# Autodesk Inventor assembly: entero
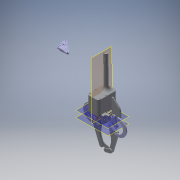
[picture p0: Inventor's stored thumbnail of the model, 180x180]
Saved by Autodesk Inventor 2018 (Build 220112000, 112)
## iProperties
Created: 2018-05-25
Part Number: entero
Document SubType Name: Assembly
Designer: vigus
Author: vigus
## Documents named in this file (8)
- C:\Users\vigus\Documents\gihug\hecatonquiros\cad_models\accesories\gripper\entero.iam
- C:\Users\vigus\Documents\gihug\hecatonquiros\cad_models\tools\gripper\serial_model_0dof\core_attachment.ipt
- C:\Users\vigus\Documents\gihug\hecatonquiros\cad_models\accesories\gripper\Imported Components\garra_pilar\garra_pilar.ipt
- C:\Users\vigus\Documents\gihug\hecatonquiros\cad_models\tools\gripper\serial_model_0dof\ScrewActuatorGripperCenter.ipt
- C:\Users\vigus\Documents\gihug\hecatonquiros\cad_models\tools\gripper\serial_model_0dof\gripper.ipt
- C:\Users\vigus\Documents\gihug\hecatonquiros\cad_models\accesories\gripper\garra_pilar_3.ipt
- C:\Users\vigus\Documents\gihug\hecatonquiros\cad_models\accesories\gripper\barra_tri.ipt
- C:\Users\vigus\Documents\gihug\hecatonquiros\cad_models\accesories\gripper\barra_triangulo.ipt
## Components (13 placed, 7 different names)
1. core_attachment:1 — Mate:2, Mate:3, Mate:13, Mate:14, Angle:1, Mate:32, Mate:42, Mate:43, Mate:52, Mate:53, Mate:55, Mate:56, Mate:69, Mate:70, Flush:1, Flush:2
2. garra_pilar:1 — Mate:2, Mate:3, Mate:59, Mate:66
3. ScrewActuatorGripperCenter:1 — Angle:1, Mate:32, Mate:64, Mate:65, Mate:67
4. garra_pilar:2 — Mate:13, Mate:14, Mate:60, Mate:61
5. gripper:1 — Mate:54, Mate:57, Mate:62, Mate:63
6. gripper:2 — Mate:68, Mate:71
7. garra_pilar:3 — Mate:42, Mate:43, Mate:58, Mate:61
8. garra_pilar_3:2 — Mate:55, Mate:56, Mate:57
9. garra_pilar_3:3 — Mate:52, Mate:53, Mate:54
10. garra_pilar_3:4 — Mate:69, Mate:70, Mate:71
11. barra_tri:2
12. barra_triangulo:1 — Mate:58, Mate:60, Mate:62, Mate:63, Mate:64, Mate:65
13. barra_triangulo:2 — Mate:59, Mate:66, Mate:67, Mate:68
## Relationships (30: Mate 27, Flush 2, Angle 1)
- Mate:2: core_attachment:1 ↔ garra_pilar:1
- Mate:3: core_attachment:1 ↔ garra_pilar:1
- Mate:13: core_attachment:1 ↔ garra_pilar:2
- Mate:14: core_attachment:1 ↔ garra_pilar:2
- Angle:1 (0 deg): core_attachment:1 ↔ ScrewActuatorGripperCenter:1
- Mate:32: core_attachment:1 ↔ ScrewActuatorGripperCenter:1
- Mate:42: core_attachment:1 ↔ garra_pilar:3
- Mate:43: core_attachment:1 ↔ garra_pilar:3
- Mate:52: core_attachment:1 ↔ garra_pilar_3:3
- Mate:53: core_attachment:1 ↔ garra_pilar_3:3
- Mate:54: gripper:1 ↔ garra_pilar_3:3
- Mate:55: core_attachment:1 ↔ garra_pilar_3:2
- Mate:56: core_attachment:1 ↔ garra_pilar_3:2
- Mate:57: gripper:1 ↔ garra_pilar_3:2
- Mate:58: garra_pilar:3 ↔ barra_triangulo:1
- Mate:59: garra_pilar:1 ↔ barra_triangulo:2
- Mate:60: garra_pilar:2 ↔ barra_triangulo:1
- Mate:61: garra_pilar:2 ↔ garra_pilar:3
- Mate:62: gripper:1 ↔ barra_triangulo:1
- Mate:63: gripper:1 ↔ barra_triangulo:1
- Mate:64: ScrewActuatorGripperCenter:1 ↔ barra_triangulo:1
- Mate:65: ScrewActuatorGripperCenter:1 ↔ barra_triangulo:1
- Mate:66: garra_pilar:1 ↔ barra_triangulo:2
- Mate:67: ScrewActuatorGripperCenter:1 ↔ barra_triangulo:2
- Mate:68: gripper:2 ↔ barra_triangulo:2
- Mate:69: core_attachment:1 ↔ garra_pilar_3:4
- Mate:70: core_attachment:1 ↔ garra_pilar_3:4
- Mate:71: gripper:2 ↔ garra_pilar_3:4
- Flush:1 (12 mm): core_attachment:1
- Flush:2 (30 mm): core_attachment:1
